# Autodesk Inventor assembly: cup assembly
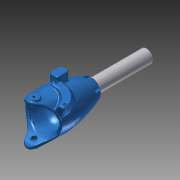
[picture p0: Inventor's stored thumbnail of the model, 180x180]
Saved by Autodesk Inventor 2015 (Build 190159000, 159)
## iProperties
Created: 2014-07-28
Part Number: cup assembly
Document SubType Name: Assembly
Designer: Jascha
Author: Jascha
## Documents named in this file (4)
- C:\Users\Jascha\Dropbox\enable\transradial arm\RIT arm\v0.43\cup assembly.iam
- C:\Users\Jascha\Dropbox\enable\transradial arm\RIT arm\v0.43\forearm cup_1.ipt
- C:\Users\Jascha\Dropbox\enable\transradial arm\RIT arm\v0.43\Retainer.ipt
- C:\Users\Jascha\Dropbox\enable\transradial arm\RIT arm\v0.43\pipe.ipt
## Components (3 placed, 3 different names)
1. forearm cup_1:1 — Mate:2, Mate:3
2. Retainer:1 — Mate:1, Mate:2
3. pipe:1 — Mate:1, Mate:3
## Relationships (3: Mate 3)
- Mate:1: Retainer:1 ↔ pipe:1
- Mate:2: forearm cup_1:1 ↔ Retainer:1
- Mate:3: forearm cup_1:1 ↔ pipe:1
